# Autodesk Inventor assembly: sprocket7_plastictips
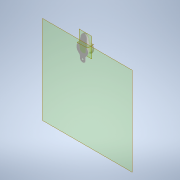
[picture p0: Inventor's stored thumbnail of the model, 180x180]
Saved by Autodesk Inventor 2020 (Build 240168000, 168)
## iProperties
Created: 2019-08-05
Part Number: sprocket7_plastictips
Document SubType Name: Assembly
Designer: erwin
Author: erwin
## Documents named in this file (4)
- D:\GitHub\BeachMaid\platform\sprocket7_plastictips.iam
- D:\GitHub\BeachMaid\platform\sprocket7_mk2.ipt
- D:\GitHub\BeachMaid\platform\sprocket7_mk2_tips.ipt
- D:\GitHub\BeachMaid\platform\sprocket7.ipt
## Components (3 placed, 3 different names)
1. sprocket7_mk2:1 — Flush:1, Flush:2, Flush:3, Flush:4
2. sprocket7_mk2_tips:1 — Flush:1, Flush:2
3. sprocket7:1 — Flush:3, Flush:4
## Relationships (4: Flush 4)
- Flush:1: sprocket7_mk2:1 ↔ sprocket7_mk2_tips:1
- Flush:2: sprocket7_mk2:1 ↔ sprocket7_mk2_tips:1
- Flush:3: sprocket7_mk2:1 ↔ sprocket7:1
- Flush:4: sprocket7_mk2:1 ↔ sprocket7:1
